# Autodesk Inventor assembly: ilmbt_3d_v1
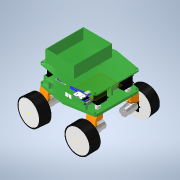
[picture p0: Inventor's stored thumbnail of the model, 180x180]
Saved by Autodesk Inventor 2021 (Build 250183000, 183)
## iProperties
Created: 2021-11-22
Part Number: ilmbt_3d_v1
Document SubType Name: Assembly
Designer: techv
Author: techv
## Documents named in this file (25)
- D:\Projects\P_Intelligent Line Marking Bot\Design\ilmbt_3d_v1\ilmbt_3d_v1.iam
- D:\Projects\P_Intelligent Line Marking Bot\Design\ilmbt_3d_v1\3d printing workspace.ipt
- D:\Projects\P_Intelligent Line Marking Bot\Design\ilmbt_3d_v1\base_.ipt
- D:\Projects\P_Intelligent Line Marking Bot\Design\LMBOT V3 80%\MG-958 servo_MIR.iam
- D:\Projects\P_Intelligent Line Marking Bot\Design\LMBOT V3 80%\knucle_MIR1.ipt
- D:\Projects\P_Intelligent Line Marking Bot\Design\LMBOT V3 80%\Symmetry of JGB37-520_MIR1.iam
- D:\Projects\P_Intelligent Line Marking Bot\Design\LMBOT V3 80%\wheel_MIR_MIR.ipt
- D:\Projects\P_Intelligent Line Marking Bot\Design\ilmbt_3d_v1\servo_shaft.ipt
- D:\Projects\P_Intelligent Line Marking Bot\Design\ilmbt_3d_v1\servo shaft flange.ipt
- D:\Projects\P_Intelligent Line Marking Bot\Design\ilmbt_3d_v1\servo flange.ipt
- C:\Users\techv\Documents\C drive Inventor Files\motor driver.ipt
- C:\Users\techv\Downloads\LM2596 DC-DC StepDown Converter v1.iam
- D:\Projects\P_Intelligent Line Marking Bot\Design\3D cad xrobot version\my designs\battery.ipt
- D:\Projects\A_Electronics CAD model\ublox-gps-1.snapshot.1\gps\parts\GPS_ublox_board.ipt
- C:\Users\techv\Documents\HCM5883L.ipt
- D:\Projects\A_Electronics CAD model\arduino-mega-atmega-2560-1.snapshot.3\Arduino Mega ATmega 2560.iam
- D:\Projects\A_Electronics CAD model\mpu-9250-9dof-imu-1.snapshot.4\MPU-9250.iam
- D:\Projects\A_Electronics CAD model\Raspberry Pi.ipt
- D:\Projects\P_Intelligent Line Marking Bot\Design\ilmbt_3d_v1\upper base.ipt
- D:\Projects\P_Intelligent Line Marking Bot\Design\ilmbt_3d_v1\ilmbt_3d_v1\AIP\FEA\dsofer334.fins
- D:\Projects\P_Intelligent Line Marking Bot\Design\ilmbt_3d_v1\ilmbt_3d_v1\AIP\FEA\dsofer334.fsat
- D:\Projects\P_Intelligent Line Marking Bot\Design\ilmbt_3d_v1\ilmbt_3d_v1\AIP\FEA\dsofer340.ftes
- D:\Projects\P_Intelligent Line Marking Bot\Design\ilmbt_3d_v1\ilmbt_3d_v1\AIP\FEA\dsofer340.fwiz
- D:\Projects\P_Intelligent Line Marking Bot\Design\ilmbt_3d_v1\ilmbt_3d_v1\AIP\FEA\dsofer36o.fmsh
- D:\Projects\P_Intelligent Line Marking Bot\Design\ilmbt_3d_v1\ilmbt_3d_v1\AIP\FEA\dsofer36p.fres
## Components (44 placed, 18 different names)
1. 3d printing workspace:1
2. base_:1 — Mate:13, Mate:14, Angle:2, Mate:15, Mate:18, Mate:22, Angle:3, Mate:24, Mate:25, Mate:26, Mate:60, Mate:61, Mate:66, Mate:68, Mate:69, Mate:70, Mate:90, Flush:43, Mate:91, Mate:92, Flush:44, Flush:45, Flush:47, Mate:93, Mate:94, Mate:95, Mate:97, Mate:98, Mate:99, Mate:109, Flush:56, Flush:57, Mate:111, Flush:60, Flush:61
3. MG-958 servo_MIR:2 [sub-assembly] — Angle:2, Mate:15, Flush:51, Flush:52, Flush:53, Flush:54
4. MG-958 servo_MIR:3 [sub-assembly] — Flush:49, Flush:50, Flush:55
5. MG-958 servo_MIR:4 [sub-assembly] — Flush:53, Flush:54, Flush:55
6. MG-958 servo_MIR:5 [sub-assembly] — Mate:17, Angle:3, Mate:23, Mate:94, Mate:95, Flush:49, Flush:50, Flush:51, Flush:52
7. knucle_MIR1:1 — Mate:8, Mate:9, Mate:10, Mate:13, Mate:14, Flush:5, Mate:21, Flush:6
8. Symmetry of JGB37-520_MIR1:1 [sub-assembly] — Mate:8, Mate:9, Mate:10, Mate:11, Mate:12
9. servo_shaft:1 — Flush:5, Mate:17, Mate:18, Mate:21, Flush:6
10. servo shaft flange:1
11. servo flange:1
12. motor driver:1 — Mate:22, Mate:23, Flush:8, Flush:12
13. motor driver:2 — Mate:24, Flush:12, Flush:13, Mate:90, Flush:43
14. motor driver:3 — Mate:25, Flush:13, Flush:14
15. motor driver:4 — Mate:26, Flush:8, Flush:14, Mate:91
16. LM2596 DC-DC StepDown Converter v1:1 [sub-assembly] — Mate:87, Flush:38, Flush:44
17. battery:1 — Flush:58, Flush:59, Mate:110
18. battery:2 — Mate:87, Mate:92, Flush:47, Mate:93, Flush:58, Flush:59, Mate:110
19. knucle_MIR1:2
20. Symmetry of JGB37-520_MIR1:2 [sub-assembly]
21. servo_shaft:2 — Mate:58, Mate:59, Mate:60, Mate:61
22. servo shaft flange:2 — Mate:55, Mate:56, Mate:57, Mate:58, Mate:59
23. servo flange:2 — Mate:55, Mate:56, Mate:57
24. knucle_MIR1:3
25. Symmetry of JGB37-520_MIR1:3 [sub-assembly]
26. wheel_MIR_MIR:1 — Mate:11, Mate:12
27. wheel_MIR_MIR:2
28. wheel_MIR_MIR:3
29. wheel_MIR_MIR:4
30. servo_shaft:3 — Mate:62, Flush:22, Mate:70
31. servo shaft flange:3 — Flush:23, Mate:71, Mate:72, Mate:73, Mate:74
32. servo flange:3 — Mate:72, Mate:73, Mate:74
33. knucle_MIR1:4
34. Symmetry of JGB37-520_MIR1:4 [sub-assembly]
35. servo_shaft:4 — Mate:68, Mate:69, Flush:23, Mate:71
36. servo shaft flange:4 — Mate:62, Flush:22, Mate:63, Mate:64, Mate:65, Mate:66
37. servo flange:4 — Mate:63, Mate:64, Mate:65
38. GPS_ublox_board:1 — Flush:39, Mate:102, Mate:108
39. HCM5883L:1 — Mate:107, Mate:108
40. Arduino Mega ATmega 2560:1 [sub-assembly] — Mate:111, Flush:60, Flush:61
41. MPU-9250:1 [sub-assembly] — Flush:39, Mate:103, Mate:105
42. Raspberry Pi:1 — Mate:109, Flush:56, Flush:57
43. LM2596 DC-DC StepDown Converter v1:2 [sub-assembly] — Flush:38, Flush:45
44. upper base:1 — Mate:97, Mate:98, Mate:99, Mate:102, Mate:103, Mate:105, Mate:107
## Relationships (106: Mate 71, Flush 33, Angle 2)
- Mate:8: knucle_MIR1:1 ↔ Symmetry of JGB37-520_MIR1:1
- Mate:9: knucle_MIR1:1 ↔ Symmetry of JGB37-520_MIR1:1
- Mate:10: knucle_MIR1:1 ↔ Symmetry of JGB37-520_MIR1:1
- Mate:11: Symmetry of JGB37-520_MIR1:1 ↔ wheel_MIR_MIR:1
- Mate:12 (10 mm): Symmetry of JGB37-520_MIR1:1 ↔ wheel_MIR_MIR:1
- Mate:13 (20 mm): base_:1 ↔ knucle_MIR1:1
- Mate:14 (40 mm): base_:1 ↔ knucle_MIR1:1
- Flush:5: knucle_MIR1:1 ↔ servo_shaft:1
- Angle:2 (0 deg): base_:1 ↔ MG-958 servo_MIR:2
- Mate:15: base_:1 ↔ MG-958 servo_MIR:2
- Mate:17: MG-958 servo_MIR:5 ↔ servo_shaft:1
- Mate:18: base_:1 ↔ servo_shaft:1
- Mate:21: knucle_MIR1:1 ↔ servo_shaft:1
- Flush:6: knucle_MIR1:1 ↔ servo_shaft:1
- Mate:22: base_:1 ↔ motor driver:1
- Angle:3 (0 deg): base_:1 ↔ MG-958 servo_MIR:5
- Mate:23 (15 mm): MG-958 servo_MIR:5 ↔ motor driver:1
- Mate:24: base_:1 ↔ motor driver:2
- Mate:25: base_:1 ↔ motor driver:3
- Mate:26: base_:1 ↔ motor driver:4
- Flush:8: motor driver:1 ↔ motor driver:4
- Flush:12: motor driver:1 ↔ motor driver:2
- Flush:13: motor driver:2 ↔ motor driver:3
- Flush:14: motor driver:3 ↔ motor driver:4
- [Mate]: knucle_MIR1:2 ↔ Symmetry of JGB37-520_MIR1:2
- [Mate]: knucle_MIR1:2 ↔ Symmetry of JGB37-520_MIR1:2
- [Mate]: knucle_MIR1:2 ↔ Symmetry of JGB37-520_MIR1:2
- [Mate]: Symmetry of JGB37-520_MIR1:2 ↔ wheel_MIR_MIR:2
- [Mate] (10 mm): Symmetry of JGB37-520_MIR1:2 ↔ wheel_MIR_MIR:2
- [Flush]: knucle_MIR1:2 ↔ servo_shaft:2
- [Mate]: knucle_MIR1:2 ↔ servo_shaft:2
- [Flush]: knucle_MIR1:2 ↔ servo_shaft:2
- [Mate]: knucle_MIR1:3 ↔ Symmetry of JGB37-520_MIR1:3
- [Mate]: knucle_MIR1:3 ↔ Symmetry of JGB37-520_MIR1:3
- [Mate]: knucle_MIR1:3 ↔ Symmetry of JGB37-520_MIR1:3
- [Mate]: Symmetry of JGB37-520_MIR1:3 ↔ wheel_MIR_MIR:3
- [Mate] (10 mm): Symmetry of JGB37-520_MIR1:3 ↔ wheel_MIR_MIR:3
- [Flush]: knucle_MIR1:3 ↔ servo_shaft:3
- [Mate]: knucle_MIR1:3 ↔ servo_shaft:3
- [Flush]: knucle_MIR1:3 ↔ servo_shaft:3
- [Mate]: knucle_MIR1:4 ↔ Symmetry of JGB37-520_MIR1:4
- [Mate]: knucle_MIR1:4 ↔ Symmetry of JGB37-520_MIR1:4
- [Mate]: knucle_MIR1:4 ↔ Symmetry of JGB37-520_MIR1:4
- [Mate]: wheel_MIR_MIR:4 ↔ Symmetry of JGB37-520_MIR1:4
- [Mate] (10 mm): wheel_MIR_MIR:4 ↔ Symmetry of JGB37-520_MIR1:4
- [Flush]: knucle_MIR1:4 ↔ servo_shaft:4
- [Mate]: knucle_MIR1:4 ↔ servo_shaft:4
- [Flush]: knucle_MIR1:4 ↔ servo_shaft:4
- Mate:55: servo shaft flange:2 ↔ servo flange:2
- Mate:56: servo shaft flange:2 ↔ servo flange:2
- Mate:57: servo shaft flange:2 ↔ servo flange:2
- Mate:58: servo_shaft:2 ↔ servo shaft flange:2
- Mate:59: servo_shaft:2 ↔ servo shaft flange:2
- Mate:60: base_:1 ↔ servo_shaft:2
- Mate:61: base_:1 ↔ servo_shaft:2
- Mate:62: servo_shaft:3 ↔ servo shaft flange:4
- Flush:22: servo_shaft:3 ↔ servo shaft flange:4
- Mate:63: servo shaft flange:4 ↔ servo flange:4
- Mate:64: servo shaft flange:4 ↔ servo flange:4
- Mate:65: servo shaft flange:4 ↔ servo flange:4
- Mate:66: base_:1 ↔ servo shaft flange:4
- Mate:68: base_:1 ↔ servo_shaft:4
- Mate:69: base_:1 ↔ servo_shaft:4
- Mate:70: base_:1 ↔ servo_shaft:3
- Flush:23: servo shaft flange:3 ↔ servo_shaft:4
- Mate:71: servo shaft flange:3 ↔ servo_shaft:4
- Mate:72: servo shaft flange:3 ↔ servo flange:3
- Mate:73: servo shaft flange:3 ↔ servo flange:3
- Mate:74: servo shaft flange:3 ↔ servo flange:3
- Mate:87 (15 mm): LM2596 DC-DC StepDown Converter v1:1 ↔ battery:2
- Flush:38: LM2596 DC-DC StepDown Converter v1:1 ↔ LM2596 DC-DC StepDown Converter v1:2
- Flush:39: GPS_ublox_board:1 ↔ MPU-9250:1
- Mate:90: base_:1 ↔ motor driver:2
- Flush:43: base_:1 ↔ motor driver:2
- Mate:91: base_:1 ↔ motor driver:4
- Mate:92: base_:1 ↔ battery:2
- Flush:44 (15 mm): base_:1 ↔ LM2596 DC-DC StepDown Converter v1:1
- Flush:45 (15 mm): base_:1 ↔ LM2596 DC-DC StepDown Converter v1:2
- Flush:47 (20 mm): base_:1 ↔ battery:2
- Mate:93 (25 mm): base_:1 ↔ battery:2
- Mate:94: base_:1 ↔ MG-958 servo_MIR:5
- Mate:95: base_:1 ↔ MG-958 servo_MIR:5
- Flush:49: MG-958 servo_MIR:3 ↔ MG-958 servo_MIR:5
- Flush:50: MG-958 servo_MIR:3 ↔ MG-958 servo_MIR:5
- Flush:51: MG-958 servo_MIR:2 ↔ MG-958 servo_MIR:5
- Flush:52: MG-958 servo_MIR:2 ↔ MG-958 servo_MIR:5
- Flush:53: MG-958 servo_MIR:2 ↔ MG-958 servo_MIR:4
- Flush:54: MG-958 servo_MIR:2 ↔ MG-958 servo_MIR:4
- Flush:55: MG-958 servo_MIR:3 ↔ MG-958 servo_MIR:4
- Mate:97: base_:1 ↔ upper base:1
- Mate:98: base_:1 ↔ upper base:1
- Mate:99 (70 mm): base_:1 ↔ upper base:1
- Mate:102 (3 mm): GPS_ublox_board:1 ↔ upper base:1
- Mate:103 (3 mm): MPU-9250:1 ↔ upper base:1
- Mate:105 (3 mm): MPU-9250:1 ↔ upper base:1
- Mate:107 (3 mm): HCM5883L:1 ↔ upper base:1
- Mate:108 (5 mm): GPS_ublox_board:1 ↔ HCM5883L:1
- Mate:109 (3 mm): base_:1 ↔ Raspberry Pi:1
- Flush:56: base_:1 ↔ Raspberry Pi:1
- Flush:57 (3 mm): base_:1 ↔ Raspberry Pi:1
- Flush:58: battery:1 ↔ battery:2
- Flush:59: battery:1 ↔ battery:2
- Mate:110: battery:1 ↔ battery:2
- Mate:111 (3 mm): base_:1 ↔ Arduino Mega ATmega 2560:1
- Flush:60: base_:1 ↔ Arduino Mega ATmega 2560:1
- Flush:61 (3 mm): base_:1 ↔ Arduino Mega ATmega 2560:1
## Named parameters: sa_0 = 1000, d72_d43 = 0 mm, d73_d44 = 0 mm, d74_d25 = 0 mm, d75_d26 = 0 mm, d76_d27 = 0 mm, d77_d28 = 0 mm, d78_d29 = 10 mm, d79_d32 = 0 mm, d80_d43 = 0 mm, d81_d44 = 0 mm, d82_d25 = 0 mm, d83_d26 = 0 mm, d84_d27 = 0 mm, d85_d28 = 0 mm, d86_d29 = 10 mm, d87_d32 = 0 mm, d88_d43 = 0 mm, d89_d44 = 0 mm, d90_d25 = 0 mm, d91_d26 = 0 mm, d92_d27 = 0 mm, d93_d28 = 0 mm, d94_d29 = 10 mm, d95_d32 = 0 mm
note: some values were not read from the file. Shown as the stored number, unit unknown: "sa_0".
